# Autodesk Inventor assembly: testLift
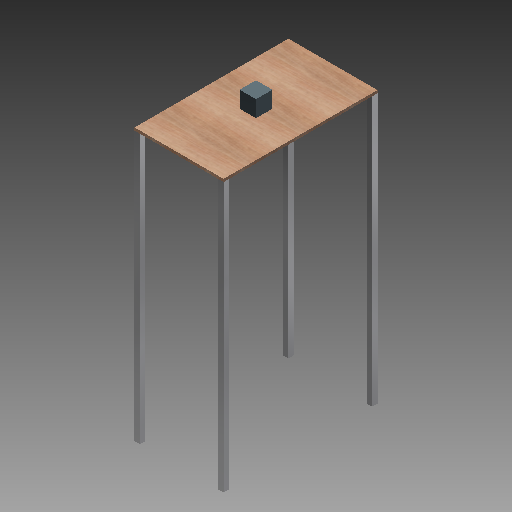
[picture p0: Inventor's stored thumbnail of the model, 512x512]
Saved by Autodesk Inventor 2018.2 (Build 222227000, 227)
## iProperties
Created: 2018-01-07
Part Number: testLift
Document SubType Name: Assembly
Designer: steele
Mass: 10943.7 g
Surface Area: 15572.6 cm^2
Volume: 5612.36 cm^3
Density: 1.94992 g/cm^3
Author: steele
## Documents named in this file (4)
- D:\snobotics\CAD-Development\robSteele\2018-FRC\LiftCubeManipulator\testLift.iam
- D:\snobotics\CAD-Development\robSteele\2018-FRC\LiftCubeManipulator\plywoodBase.ipt
- D:\snobotics\CAD-Development\robSteele\2018-FRC\LiftCubeManipulator\supportForLift.ipt
- D:\snobotics\CAD-Development\robSteele\2018-FRC\LiftCubeManipulator\sampleWeight.ipt
## Components (3 placed, 3 different names)
1. plywoodBase:1 — Mate:1, Flush:1, Flush:2, Mate:2, Mate:3, Mate:4
2. supportForLift:1 — Mate:1, Flush:1, Flush:2
3. sampleWeight:1 — Mate:2, Mate:3, Mate:4
## Relationships (6: Mate 4, Flush 2)
- Mate:1: plywoodBase:1 ↔ supportForLift:1
- Flush:1: plywoodBase:1 ↔ supportForLift:1
- Flush:2: plywoodBase:1 ↔ supportForLift:1
- Mate:2: plywoodBase:1 ↔ sampleWeight:1
- Mate:3: plywoodBase:1 ↔ sampleWeight:1
- Mate:4: plywoodBase:1 ↔ sampleWeight:1
